# Autodesk Inventor assembly: KosselCNC
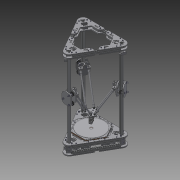
[picture p0: Inventor's stored thumbnail of the model, 180x180]
Saved by Autodesk Inventor 2014 (Build 180170000, 170)
## iProperties
Created: 2014-08-25
Part Number: KosselCNC
Document SubType Name: Assembly
Designer: ThatOtherGuy
Author: ThatOtherGuy
## Documents named in this file (10)
- C:\Users\ThatOtherGuy\Documents\Inventor\KosselCNC\KosselCNC.iam
- C:\Users\ThatOtherGuy\Documents\Inventor\KosselCNC\Frame\KosselCNC1515_Vertex_Lower.iam
- C:\Users\ThatOtherGuy\Documents\Inventor\KosselCNC\Rail_Misumi_HFS3-1515-600.ipt
- C:\Users\ThatOtherGuy\Documents\Inventor\KosselCNC\Carriage\Carriage.iam
- C:\Users\ThatOtherGuy\Documents\Inventor\KosselCNC\Effector\Effector.iam
- C:\Users\ThatOtherGuy\Documents\Inventor\KosselCNC\Frame\KosselCNC1515_Vertex_Upper.iam
- C:\Users\ThatOtherGuy\Documents\Inventor\KosselCNC\Frame\EndStop.iam
- C:\Users\ThatOtherGuy\Documents\Inventor\KosselCNC\Effector\Effector_Arm.iam
- C:\Users\ThatOtherGuy\Documents\Inventor\KosselCNC\Rail_Misumi_HFS3-1515-240.ipt
- C:\Users\ThatOtherGuy\Documents\Inventor\KosselCNC\Frame\Bed.iam
## Components (32 placed, 9 different names)
1. Bed:1 [sub-assembly] — Mate:38, Mate:39, Mate:40, Mate:41
2. Effector:1 [sub-assembly] — Tangent:39, Tangent:46, Tangent:47, Tangent:41, Tangent:45, Tangent:44, Mate:41
3. KosselCNC1515_Vertex_Lower:1 [sub-assembly] — Flush:1, Flush:2, Mate:2, Flush:3, Tangent:3, Tangent:4, Mate:7, Mate:12, Mate:13, Flush:14, Mate:38, Mate:39
4. Rail_Misumi_HFS3-1515-240:1 — Mate:2, Flush:3, Tangent:1, Tangent:4, Flush:8, Flush:9
5. Rail_Misumi_HFS3-1515-240:4 — Flush:8, Flush:9, Mate:7
6. KosselCNC1515_Vertex_Lower:2 [sub-assembly] — Flush:1, Flush:2, Tangent:1, Flush:4, Flush:5, Tangent:5, Mate:9, Flush:16, Mate:14, Mate:15
7. Rail_Misumi_HFS3-1515-240:2 — Mate:4, Flush:7, Tangent:2, Tangent:5, Flush:10, Flush:11
8. Rail_Misumi_HFS3-1515-240:5 — Flush:10, Flush:11, Mate:9
9. KosselCNC1515_Vertex_Lower:3 [sub-assembly] — Flush:4, Flush:5, Mate:4, Mate:5, Flush:6, Flush:7, Tangent:2, Mate:8, Flush:15, Mate:16, Mate:17
10. Rail_Misumi_HFS3-1515-240:3 — Mate:5, Flush:6, Tangent:3, Flush:12, Flush:13
11. Rail_Misumi_HFS3-1515-240:6 — Flush:12, Flush:13, Mate:8, Mate:40
12. Effector_Arm:1 [sub-assembly] — Tangent:38, Tangent:39
13. Effector_Arm:2 [sub-assembly] — Tangent:40, Tangent:41
14. Carriage:1 [sub-assembly] — Tangent:10, Tangent:11, Tangent:12, Tangent:38, Tangent:40, Flush:30, Flush:31
15. Effector_Arm:3 [sub-assembly] — Tangent:42, Tangent:45
16. Effector_Arm:4 [sub-assembly] — Tangent:43, Tangent:44
17. Carriage:2 [sub-assembly] — Tangent:13, Tangent:14, Tangent:15, Tangent:42, Tangent:43, Flush:30
18. Effector_Arm:5 [sub-assembly] — Tangent:49, Tangent:46
19. Effector_Arm:6 [sub-assembly] — Tangent:48, Tangent:47
20. Carriage:3 [sub-assembly] — Tangent:16, Tangent:17, Tangent:18, Tangent:48, Tangent:49, Flush:31
21. Rail_Misumi_HFS3-1515-600:1 — Mate:12, Mate:13, Flush:14, Tangent:10, Tangent:11, Tangent:12, Mate:18, Mate:19, Flush:19, Mate:28, Mate:29
22. Rail_Misumi_HFS3-1515-600:2 — Flush:16, Mate:14, Mate:15, Tangent:13, Tangent:14, Tangent:15, Mate:34, Tangent:54
23. Rail_Misumi_HFS3-1515-600:3 — Flush:15, Mate:16, Mate:17, Tangent:16, Tangent:17, Tangent:18, Mate:37, Tangent:55
24. EndStop:1 [sub-assembly] — Mate:28, Mate:29, Mate:31
25. KosselCNC1515_Vertex_Upper:1 [sub-assembly] — Mate:18, Mate:19, Flush:19, Mate:20, Flush:20, Tangent:31, Mate:31
26. Rail_Misumi_HFS3-1515-240:7 — Mate:20, Flush:20, Tangent:31, Mate:21, Flush:21, Tangent:32
27. EndStop:2 [sub-assembly] — Mate:34, Tangent:54, Mate:35
28. KosselCNC1515_Vertex_Upper:2 [sub-assembly] — Mate:21, Flush:21, Tangent:32, Tangent:33, Flush:22, Mate:22, Mate:35
29. Rail_Misumi_HFS3-1515-240:8 — Tangent:33, Flush:22, Mate:22, Mate:23, Flush:23, Tangent:34
30. EndStop:3 [sub-assembly] — Mate:36, Mate:37, Tangent:55
31. KosselCNC1515_Vertex_Upper:3 [sub-assembly] — Mate:23, Flush:23, Tangent:34, Tangent:35, Flush:24, Mate:24, Mate:36
32. Rail_Misumi_HFS3-1515-240:9 — Tangent:35, Flush:24, Mate:24
## Relationships (87: Tangent 33, Mate 30, Flush 24)
- Flush:1: KosselCNC1515_Vertex_Lower:1 ↔ KosselCNC1515_Vertex_Lower:2
- Flush:2: KosselCNC1515_Vertex_Lower:1 ↔ KosselCNC1515_Vertex_Lower:2
- Mate:2: KosselCNC1515_Vertex_Lower:1 ↔ Rail_Misumi_HFS3-1515-240:1
- Flush:3: KosselCNC1515_Vertex_Lower:1 ↔ Rail_Misumi_HFS3-1515-240:1
- Tangent:1: Rail_Misumi_HFS3-1515-240:1 ↔ KosselCNC1515_Vertex_Lower:2
- Flush:4: KosselCNC1515_Vertex_Lower:2 ↔ KosselCNC1515_Vertex_Lower:3
- Flush:5: KosselCNC1515_Vertex_Lower:2 ↔ KosselCNC1515_Vertex_Lower:3
- Mate:4: Rail_Misumi_HFS3-1515-240:2 ↔ KosselCNC1515_Vertex_Lower:3
- Mate:5: KosselCNC1515_Vertex_Lower:3 ↔ Rail_Misumi_HFS3-1515-240:3
- Flush:6: KosselCNC1515_Vertex_Lower:3 ↔ Rail_Misumi_HFS3-1515-240:3
- Flush:7: Rail_Misumi_HFS3-1515-240:2 ↔ KosselCNC1515_Vertex_Lower:3
- Tangent:2: Rail_Misumi_HFS3-1515-240:2 ↔ KosselCNC1515_Vertex_Lower:3
- Tangent:3: KosselCNC1515_Vertex_Lower:1 ↔ Rail_Misumi_HFS3-1515-240:3
- Tangent:4: KosselCNC1515_Vertex_Lower:1 ↔ Rail_Misumi_HFS3-1515-240:1
- Tangent:5: KosselCNC1515_Vertex_Lower:2 ↔ Rail_Misumi_HFS3-1515-240:2
- Flush:8: Rail_Misumi_HFS3-1515-240:1 ↔ Rail_Misumi_HFS3-1515-240:4
- Flush:9: Rail_Misumi_HFS3-1515-240:1 ↔ Rail_Misumi_HFS3-1515-240:4
- Mate:7: KosselCNC1515_Vertex_Lower:1 ↔ Rail_Misumi_HFS3-1515-240:4
- Flush:10: Rail_Misumi_HFS3-1515-240:2 ↔ Rail_Misumi_HFS3-1515-240:5
- Flush:11: Rail_Misumi_HFS3-1515-240:2 ↔ Rail_Misumi_HFS3-1515-240:5
- Flush:12: Rail_Misumi_HFS3-1515-240:3 ↔ Rail_Misumi_HFS3-1515-240:6
- Flush:13: Rail_Misumi_HFS3-1515-240:3 ↔ Rail_Misumi_HFS3-1515-240:6
- Mate:8: KosselCNC1515_Vertex_Lower:3 ↔ Rail_Misumi_HFS3-1515-240:6
- Mate:9: KosselCNC1515_Vertex_Lower:2 ↔ Rail_Misumi_HFS3-1515-240:5
- Mate:12: KosselCNC1515_Vertex_Lower:1 ↔ Rail_Misumi_HFS3-1515-600:1
- Mate:13: KosselCNC1515_Vertex_Lower:1 ↔ Rail_Misumi_HFS3-1515-600:1
- Flush:14: KosselCNC1515_Vertex_Lower:1 ↔ Rail_Misumi_HFS3-1515-600:1
- Flush:15: KosselCNC1515_Vertex_Lower:3 ↔ Rail_Misumi_HFS3-1515-600:3
- Flush:16: KosselCNC1515_Vertex_Lower:2 ↔ Rail_Misumi_HFS3-1515-600:2
- Mate:14: KosselCNC1515_Vertex_Lower:2 ↔ Rail_Misumi_HFS3-1515-600:2
- Mate:15: KosselCNC1515_Vertex_Lower:2 ↔ Rail_Misumi_HFS3-1515-600:2
- Mate:16: KosselCNC1515_Vertex_Lower:3 ↔ Rail_Misumi_HFS3-1515-600:3
- Mate:17: KosselCNC1515_Vertex_Lower:3 ↔ Rail_Misumi_HFS3-1515-600:3
- Tangent:10: Carriage:1 ↔ Rail_Misumi_HFS3-1515-600:1
- Tangent:11: Carriage:1 ↔ Rail_Misumi_HFS3-1515-600:1
- Tangent:12: Carriage:1 ↔ Rail_Misumi_HFS3-1515-600:1
- Tangent:13: Carriage:2 ↔ Rail_Misumi_HFS3-1515-600:2
- Tangent:14: Carriage:2 ↔ Rail_Misumi_HFS3-1515-600:2
- Tangent:15: Carriage:2 ↔ Rail_Misumi_HFS3-1515-600:2
- Tangent:16: Carriage:3 ↔ Rail_Misumi_HFS3-1515-600:3
- Tangent:17: Carriage:3 ↔ Rail_Misumi_HFS3-1515-600:3
- Tangent:18: Carriage:3 ↔ Rail_Misumi_HFS3-1515-600:3
- Mate:18: Rail_Misumi_HFS3-1515-600:1 ↔ KosselCNC1515_Vertex_Upper:1
- Mate:19: Rail_Misumi_HFS3-1515-600:1 ↔ KosselCNC1515_Vertex_Upper:1
- Flush:19: Rail_Misumi_HFS3-1515-600:1 ↔ KosselCNC1515_Vertex_Upper:1
- Mate:20: KosselCNC1515_Vertex_Upper:1 ↔ Rail_Misumi_HFS3-1515-240:7
- Flush:20: KosselCNC1515_Vertex_Upper:1 ↔ Rail_Misumi_HFS3-1515-240:7
- Tangent:31: KosselCNC1515_Vertex_Upper:1 ↔ Rail_Misumi_HFS3-1515-240:7
- Mate:21: Rail_Misumi_HFS3-1515-240:7 ↔ KosselCNC1515_Vertex_Upper:2
- Flush:21: Rail_Misumi_HFS3-1515-240:7 ↔ KosselCNC1515_Vertex_Upper:2
- Tangent:32: Rail_Misumi_HFS3-1515-240:7 ↔ KosselCNC1515_Vertex_Upper:2
- Tangent:33: KosselCNC1515_Vertex_Upper:2 ↔ Rail_Misumi_HFS3-1515-240:8
- Flush:22: KosselCNC1515_Vertex_Upper:2 ↔ Rail_Misumi_HFS3-1515-240:8
- Mate:22: KosselCNC1515_Vertex_Upper:2 ↔ Rail_Misumi_HFS3-1515-240:8
- Mate:23: Rail_Misumi_HFS3-1515-240:8 ↔ KosselCNC1515_Vertex_Upper:3
- Flush:23: Rail_Misumi_HFS3-1515-240:8 ↔ KosselCNC1515_Vertex_Upper:3
- Tangent:34: Rail_Misumi_HFS3-1515-240:8 ↔ KosselCNC1515_Vertex_Upper:3
- Tangent:35: KosselCNC1515_Vertex_Upper:3 ↔ Rail_Misumi_HFS3-1515-240:9
- Flush:24: KosselCNC1515_Vertex_Upper:3 ↔ Rail_Misumi_HFS3-1515-240:9
- Mate:24: KosselCNC1515_Vertex_Upper:3 ↔ Rail_Misumi_HFS3-1515-240:9
- Mate:28: Rail_Misumi_HFS3-1515-600:1 ↔ EndStop:1
- Mate:29 (1.7 mm): Rail_Misumi_HFS3-1515-600:1 ↔ EndStop:1
- Tangent:38: Effector_Arm:1 ↔ Carriage:1
- Tangent:39: Effector:1 ↔ Effector_Arm:1
- Tangent:40: Effector_Arm:2 ↔ Carriage:1
- Tangent:41: Effector:1 ↔ Effector_Arm:2
- Tangent:42: Effector_Arm:3 ↔ Carriage:2
- Tangent:43: Effector_Arm:4 ↔ Carriage:2
- Tangent:44: Effector:1 ↔ Effector_Arm:4
- Tangent:45: Effector:1 ↔ Effector_Arm:3
- Tangent:46: Effector:1 ↔ Effector_Arm:5
- Tangent:47: Effector:1 ↔ Effector_Arm:6
- Tangent:48: Effector_Arm:6 ↔ Carriage:3
- Tangent:49: Effector_Arm:5 ↔ Carriage:3
- Mate:31: EndStop:1 ↔ KosselCNC1515_Vertex_Upper:1
- Mate:34: Rail_Misumi_HFS3-1515-600:2 ↔ EndStop:2
- Tangent:54: Rail_Misumi_HFS3-1515-600:2 ↔ EndStop:2
- Mate:35: EndStop:2 ↔ KosselCNC1515_Vertex_Upper:2
- Mate:36: EndStop:3 ↔ KosselCNC1515_Vertex_Upper:3
- Mate:37: Rail_Misumi_HFS3-1515-600:3 ↔ EndStop:3
- Tangent:55: Rail_Misumi_HFS3-1515-600:3 ↔ EndStop:3
- Flush:30: Carriage:1 ↔ Carriage:2
- Flush:31: Carriage:1 ↔ Carriage:3
- Mate:38: Bed:1 ↔ KosselCNC1515_Vertex_Lower:1
- Mate:39: Bed:1 ↔ KosselCNC1515_Vertex_Lower:1
- Mate:40: Bed:1 ↔ Rail_Misumi_HFS3-1515-240:6
- Mate:41 (20 mm): Bed:1 ↔ Effector:1
